# Autodesk Inventor assembly: boardB
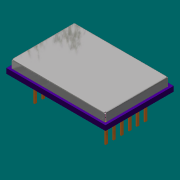
[picture p0: Inventor's stored thumbnail of the model, 180x180]
Saved by Autodesk Inventor 2016 SP1 (Build 200210100, 210)
## iProperties
Created: 2016-02-15
Part Number: boardB
Document SubType Name: Assembly
Designer: sawai
Author: sawai
## Documents named in this file (16)
- C:\Users\sawai\OneDrive\projects\mppcHighVoltage\cad\highVoltageMppc.iam
- C:\Users\sawai\OneDrive\projects\mppcHighVoltage\cad\highVoltageMppcPcb.ipt
- C:\Users\sawai\OneDrive\projects\mppcHighVoltage\cad\electronics\qfn\qfn-12.ipt
- C:\Users\Sawaiz\OneDrive\projects\highVoltageMppc\cad\electronics\qfn.ipt
- C:\Users\sawai\OneDrive\projects\mppcHighVoltage\cad\electronics\chipResistor\chipResistor-0402.ipt
- C:\Users\Sawaiz\OneDrive\projects\highVoltageMppc\cad\electronics\chipResistor.ipt
- C:\Users\sawai\OneDrive\projects\mppcHighVoltage\cad\electronics\SOT23-3.ipt
- C:\Users\sawai\OneDrive\projects\mppcHighVoltage\cad\electronics\capacitor-1206.ipt
- C:\Users\Sawaiz\OneDrive\projects\highVoltageMppc\cad\electronics\capacitor.ipt
- C:\Users\sawai\OneDrive\projects\mppcHighVoltage\cad\electronics\sod-80.ipt
- C:\Users\sawai\OneDrive\projects\mppcHighVoltage\cad\electronics\capacitor-0402.ipt
- C:\Users\sawai\OneDrive\projects\mppcHighVoltage\cad\electronics\SRN4018.ipt
- C:\Users\sawai\OneDrive\projects\mppcHighVoltage\cad\electronics\inductor-1007.ipt
- C:\Users\Sawaiz\OneDrive\projects\highVoltageMppc\cad\electronics\inductor.ipt
- C:\Users\sawai\OneDrive\projects\mppcHighVoltage\cad\electronics\S02-30200250.ipt
- C:\Users\sawai\OneDrive\projects\mppcHighVoltage\cad\electronics\2.54 Breakaway\1x6.iam
## Components (19 placed, 11 different names)
1. highVoltageMppcPcb:1 — Mate:1, Angle:1, Mate:2, Angle:6, Mate:3, Angle:7, Mate:4, Angle:11, Tangent:1, Angle:12, Mate:5, Mate:6, Angle:14, Angle:15, Mate:7, Mate:8, Angle:16, Angle:18, Angle:19, Angle:20, Mate:9, Mate:10
2. qfn-12:1 — Mate:1, Angle:1
3. chipResistor-0402:1 — Flush:1, Mate:2, Angle:4, Angle:5, Angle:13
4. chipResistor-0402:2 — Flush:1, Flush:2, Angle:3, Angle:4
5. chipResistor-0402:3 — Flush:2, Flush:3, Flush:4, Angle:2, Angle:3
6. chipResistor-0402:4 — Flush:3, Angle:2
7. chipResistor-0402:5 — Flush:4, Angle:5, Angle:6
8. SOT23-3:1 — Mate:3, Angle:7
9. capacitor-1206:1 — Flush:5, Flush:6, Flush:7, Angle:8
10. capacitor-1206:2 — Flush:5, Angle:9, Angle:10
11. capacitor-1206:3 — Flush:6, Angle:10, Angle:11
12. capacitor-1206:4 — Flush:7, Mate:4, Angle:8, Angle:9
13. sod-80:1 — Tangent:1, Angle:12
14. capacitor-0402:5 — Angle:13, Mate:5
15. SRN4018:1 — Mate:6, Angle:14
16. inductor-1007:1 — Angle:15, Mate:7
17. S02-30200250:1 — Mate:8, Angle:16
18. 1x6:1 [sub-assembly] — Angle:17, Angle:19, Mate:10, Flush:8
19. 1x6:2 [sub-assembly] — Angle:17, Angle:18, Angle:20, Mate:9, Flush:8
## Relationships (39: Angle 20, Mate 10, Flush 8, Tangent 1)
- Mate:1: highVoltageMppcPcb:1 ↔ qfn-12:1
- Angle:1 (0 deg): highVoltageMppcPcb:1 ↔ qfn-12:1
- Flush:1: chipResistor-0402:1 ↔ chipResistor-0402:2
- Flush:2: chipResistor-0402:2 ↔ chipResistor-0402:3
- Flush:3: chipResistor-0402:3 ↔ chipResistor-0402:4
- Flush:4: chipResistor-0402:3 ↔ chipResistor-0402:5
- Mate:2: highVoltageMppcPcb:1 ↔ chipResistor-0402:1
- Angle:2 (0 deg): chipResistor-0402:3 ↔ chipResistor-0402:4
- Angle:3 (0 deg): chipResistor-0402:2 ↔ chipResistor-0402:3
- Angle:4 (0 deg): chipResistor-0402:1 ↔ chipResistor-0402:2
- Angle:5 (0 deg): chipResistor-0402:1 ↔ chipResistor-0402:5
- Angle:6 (0 deg): highVoltageMppcPcb:1 ↔ chipResistor-0402:5
- Mate:3: highVoltageMppcPcb:1 ↔ SOT23-3:1
- Angle:7 (0 deg): highVoltageMppcPcb:1 ↔ SOT23-3:1
- Flush:5: capacitor-1206:1 ↔ capacitor-1206:2
- Flush:6: capacitor-1206:1 ↔ capacitor-1206:3
- Flush:7: capacitor-1206:1 ↔ capacitor-1206:4
- Mate:4: highVoltageMppcPcb:1 ↔ capacitor-1206:4
- Angle:8 (0 deg): capacitor-1206:1 ↔ capacitor-1206:4
- Angle:9 (0 deg): capacitor-1206:2 ↔ capacitor-1206:4
- Angle:10 (0 deg): capacitor-1206:2 ↔ capacitor-1206:3
- Angle:11 (0 deg): highVoltageMppcPcb:1 ↔ capacitor-1206:3
- Tangent:1: highVoltageMppcPcb:1 ↔ sod-80:1
- Angle:12 (0 deg): highVoltageMppcPcb:1 ↔ sod-80:1
- Angle:13 (0 deg): chipResistor-0402:1 ↔ capacitor-0402:5
- Mate:5: highVoltageMppcPcb:1 ↔ capacitor-0402:5
- Mate:6: highVoltageMppcPcb:1 ↔ SRN4018:1
- Angle:14 (0 deg): highVoltageMppcPcb:1 ↔ SRN4018:1
- Angle:15 (0 deg): highVoltageMppcPcb:1 ↔ inductor-1007:1
- Mate:7: highVoltageMppcPcb:1 ↔ inductor-1007:1
- Mate:8: highVoltageMppcPcb:1 ↔ S02-30200250:1
- Angle:16 (0 deg): highVoltageMppcPcb:1 ↔ S02-30200250:1
- Angle:17 (0 deg): 1x6:1 ↔ 1x6:2
- Angle:18 (0 deg): highVoltageMppcPcb:1 ↔ 1x6:2
- Angle:19 (0 deg): highVoltageMppcPcb:1 ↔ 1x6:1
- Angle:20 (0 deg): highVoltageMppcPcb:1 ↔ 1x6:2
- Mate:9: highVoltageMppcPcb:1 ↔ 1x6:2
- Mate:10: highVoltageMppcPcb:1 ↔ 1x6:1
- Flush:8: 1x6:1 ↔ 1x6:2
